# Autodesk Inventor assembly: 4x2020_in
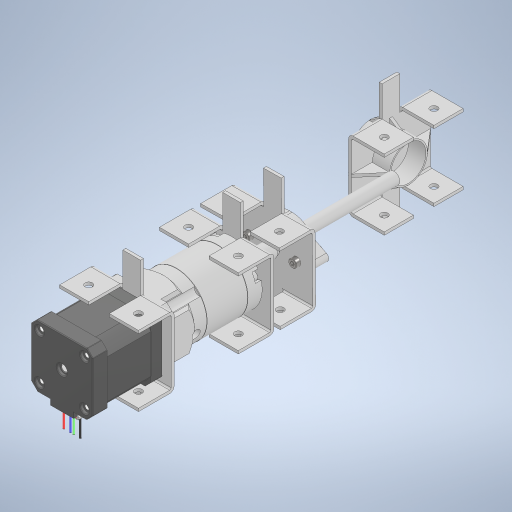
[picture p0: Inventor's stored thumbnail of the model, 512x512]
Saved by Autodesk Inventor 2024 (Build 280153000, 153)
## iProperties
Created: 2025-12-16
Part Number: 4x2020_in
Document SubType Name: Assembly
Designer: schar
Author: schar
## Documents named in this file (8)
- C:\Users\schar\Desktop\projectBlueprint\AMSTS\hardware\4x2020_in.iam
- C:\Users\schar\Desktop\projectBlueprint\AMSTS\hardware\4x2020_universal.ipt
- C:\Users\schar\Desktop\projectBlueprint\AMSTS\hardware\17HE19-2004S.ipt
- C:\Users\schar\Desktop\projectBlueprint\AMSTS\hardware\4x2020_universal_planetary.ipt
- C:\Users\schar\Desktop\projectBlueprint\AMSTS\hardware\EG17-G20.iam
- C:\Users\schar\Desktop\projectBlueprint\AMSTS\hardware\4x2020_axis.ipt
- C:\Users\schar\Desktop\projectBlueprint\AMSTS\hardware\4x2020_encoder.iam
- C:\Users\schar\Desktop\projectBlueprint\AMSTS\hardware\4x2020_axis_end_bearings.ipt
## Components (7 placed, 7 different names)
1. 4x2020_universal:1 — Mate:1, Mate:2, Mate:3, Mate:4, Mate:5, Mate:6
2. 17HE19-2004S:1 — Mate:1, Mate:2, Mate:3
3. 4x2020_universal_planetary:1 — Mate:7, Mate:8, Mate:9
4. EG17-G20:1 [sub-assembly] — Mate:4, Mate:5, Mate:6, Mate:7, Mate:8, Mate:9, Mate:10, Mate:11
5. 4x2020_axis:1 — Mate:10, Mate:11, Mate:12, Mate:13
6. 4x2020_encoder:1 [sub-assembly] — Mate:12, Mate:13
7. 4x2020_axis_end_bearings:1
## Relationships (13: Mate 13)
- Mate:1: 4x2020_universal:1 ↔ 17HE19-2004S:1
- Mate:2: 4x2020_universal:1 ↔ 17HE19-2004S:1
- Mate:3: 4x2020_universal:1 ↔ 17HE19-2004S:1
- Mate:4: 4x2020_universal:1 ↔ EG17-G20:1
- Mate:5: 4x2020_universal:1 ↔ EG17-G20:1
- Mate:6: 4x2020_universal:1 ↔ EG17-G20:1
- Mate:7: 4x2020_universal_planetary:1 ↔ EG17-G20:1
- Mate:8: 4x2020_universal_planetary:1 ↔ EG17-G20:1
- Mate:9: 4x2020_universal_planetary:1 ↔ EG17-G20:1
- Mate:10: EG17-G20:1 ↔ 4x2020_axis:1
- Mate:11: EG17-G20:1 ↔ 4x2020_axis:1
- Mate:12 (2 mm): 4x2020_axis:1 ↔ 4x2020_encoder:1
- Mate:13: 4x2020_axis:1 ↔ 4x2020_encoder:1
